# Autodesk Inventor assembly: правый привод
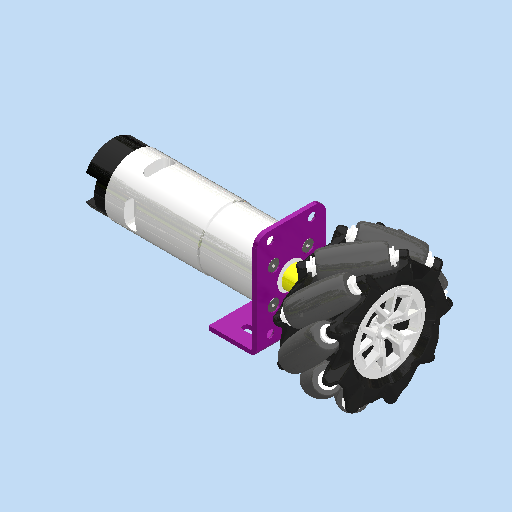
[picture p0: Inventor's stored thumbnail of the model, 512x512]
Saved by Autodesk Inventor 2025 (Build 290162000, 162)
## iProperties
Created: 2025-02-16
Part Number: правый привод
Document SubType Name: Assembly
Designer: volko
Mass: 737.749 g
Surface Area: 1037.78 cm^2
Volume: 329.761 cm^3
Density: 2.23722 g/cm^3
Author: volko
## Documents named in this file (8)
- C:\Users\volko\Desktop\диплом\Модели\детали\правый привод.iam
- C:\Users\volko\Desktop\диплом\Модели\Mecanum wheel - right\Mecanum wheel - right.iam
- C:\Users\volko\Desktop\диплом\Модели\детали\CHP-42GP-775 ABHL.ipt
- C:\Users\volko\Desktop\диплом\Модели\детали\кронштейн.ipt
- C:\Users\volko\Desktop\диплом\Модели\детали\переходная втулка.ipt
- C:\Users\volko\Desktop\диплом\Модели\детали\стандартные изделия\ru-RU\DIN 7991(2)\DIN 7991 - M4x8.ipt
- C:\Users\volko\Desktop\диплом\Модели\детали\стандартные изделия\ru-RU\DIN 913\DIN 913 - M3 x 4.ipt
- C:\Users\volko\Desktop\диплом\Модели\детали\стандартные изделия\ru-RU\ISO 7380-1\ISO 7380-1 - M4 x 25.ipt
## Components (10 placed, 7 different names)
1. Mecanum wheel - right:1 [sub-assembly] — Совмещение:8, Совмещение:9, Совмещение:10, Совмещение:20, Совмещение:21
2. CHP-42GP-775 ABHL:1 — Совмещение:1, Совмещение:2, Заподлицо:1, Совмещение:3, Совмещение:5, Совмещение:6, Совмещение:7, Совмещение:11, Совмещение:19
3. кронштейн:1 — Совмещение:3, Совмещение:5, Совмещение:11, Совмещение:13, Совмещение:14, Совмещение:15, Совмещение:16
4. переходная втулка:1 — Совмещение:6, Совмещение:7, Совмещение:8, Совмещение:9, Совмещение:10, Совмещение:17, Совмещение:18
5. DIN 913 M3 x 4:1 — Совмещение:17, Совмещение:19
6. ISO 7380-1 M4 x 25:1 — Совмещение:20, Совмещение:21
7. DIN 7991 M4x8:4 — Совмещение:16
8. DIN 7991 M4x8:3 — Совмещение:15
9. DIN 7991 M4x8:2 — Совмещение:14
10. DIN 7991 M4x8:1 — Совмещение:13
## Relationships (20: Mate 19, Flush 1)
- Совмещение:1 [Mate]: CHP-42GP-775 ABHL:1
- Совмещение:2 [Mate]: CHP-42GP-775 ABHL:1
- Заподлицо:1 [Flush]: CHP-42GP-775 ABHL:1
- Совмещение:3 [Mate]: CHP-42GP-775 ABHL:1 ↔ кронштейн:1
- Совмещение:5 [Mate]: CHP-42GP-775 ABHL:1 ↔ кронштейн:1
- Совмещение:6 [Mate]: CHP-42GP-775 ABHL:1 ↔ переходная втулка:1
- Совмещение:7 [Mate]: CHP-42GP-775 ABHL:1 ↔ переходная втулка:1
- Совмещение:8 [Mate]: Mecanum wheel - right:1 ↔ переходная втулка:1
- Совмещение:9 [Mate]: Mecanum wheel - right:1 ↔ переходная втулка:1
- Совмещение:10 [Mate]: Mecanum wheel - right:1 ↔ переходная втулка:1
- Совмещение:11 [Mate]: CHP-42GP-775 ABHL:1 ↔ кронштейн:1
- Совмещение:13 [Mate]: кронштейн:1 ↔ DIN 7991 M4x8:1
- Совмещение:14 [Mate]: кронштейн:1 ↔ DIN 7991 M4x8:2
- Совмещение:15 [Mate]: кронштейн:1 ↔ DIN 7991 M4x8:3
- Совмещение:16 [Mate]: кронштейн:1 ↔ DIN 7991 M4x8:4
- Совмещение:17 [Mate]: переходная втулка:1 ↔ DIN 913 M3 x 4:1
- Совмещение:18 [Mate]: переходная втулка:1
- Совмещение:19 [Mate]: CHP-42GP-775 ABHL:1 ↔ DIN 913 M3 x 4:1
- Совмещение:20 [Mate]: Mecanum wheel - right:1 ↔ ISO 7380-1 M4 x 25:1
- Совмещение:21 [Mate]: Mecanum wheel - right:1 ↔ ISO 7380-1 M4 x 25:1
